# Autodesk Inventor assembly: 2015 Summer Worm Drive and Bevel Gear Box for Lift
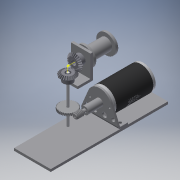
[picture p0: Inventor's stored thumbnail of the model, 180x180]
Saved by Autodesk Inventor 2016 (Build 200138000, 138)
## iProperties
Created: 2015-06-17
Part Number: 2015 Summer Worm Drive and Bevel Gear Box for Lift
Document SubType Name: Assembly
Designer: steele
Author: steele
## Documents named in this file (12)
- C:\snobotics\CAD\robSteele\Bevel Gearbox\2015 Summer Worm Drive and Bevel Gear Box for Lift.iam
- C:\snobotics\CAD\robSteele\Bevel Gearbox\baseForWormMotor.ipt
- C:\snobotics\CAD\robSteele\ipart Components\0_250 in diam aluminum rod\0_250 in diam aluminum rod-02.ipt
- C:\snobotics\CAD\robSteele\ipart Components\0_250 in diam aluminum rod.ipt
- C:\snobotics\CAD\partResources\Andy-Mark\motorMounts\AM 2488 CIM bracket.ipt
- C:\snobotics\CAD\partResources\Andy-Mark\Motors\AM 0255 MOT_CIM-Motor_217-2000.iam
- C:\snobotics\CAD\robSteele\CIM to 0_1875 Worm Gearn.ipt
- C:\snobotics\CAD\robSteele\Bevel Gearbox\g1036.ipt
- C:\snobotics\CAD\robSteele\Bevel Gearbox\LUHB.ipt
- C:\snobotics\CAD\robSteele\Bevel Gearbox\2015 Summer Bevel Gearbox\Angle Bracket for Bevel Gearbox.ipt
- C:\snobotics\CAD\robSteele\Bevel Gearbox\lift Hub.ipt
- C:\snobotics\CAD\robSteele\Bevel Gearbox\2015 Summer Bevel Gearbox\Design Accelerator\Bevel Gears1.iam
## Components (10 placed, 10 different names)
1. baseForWormMotor:1 — Insert:1, Mate:1, Flush:1, Flush:2, Insert:4
2. 0_250 in diam aluminum rod-02:1 — Insert:1, Tangent:1, Flush:3
3. AM 2488 CIM bracket:1 — Mate:1, Flush:1, Flush:2, Insert:2, Insert:3
4. AM 0255 MOT_CIM-Motor_217-2000:1 [sub-assembly] — Insert:2
5. CIM to 0_1875 Worm Gearn:1 — Insert:3, Insert:5
6. g1036:1 — Insert:4
7. LUHB:1 — Insert:5
8. Angle Bracket for Bevel Gearbox:1 — Tangent:1, Flush:3, Insert:6, Insert:7
9. lift Hub:1 — Insert:6
10. Bevel Gears:2 [sub-assembly] — Insert:7
## Relationships (12: Insert 7, Flush 3, Mate 1, Tangent 1)
- Insert:1: baseForWormMotor:1 ↔ 0_250 in diam aluminum rod-02:1
- Mate:1: baseForWormMotor:1 ↔ AM 2488 CIM bracket:1
- Flush:1: baseForWormMotor:1 ↔ AM 2488 CIM bracket:1
- Flush:2 (-101.6 mm): baseForWormMotor:1 ↔ AM 2488 CIM bracket:1
- Insert:2: AM 2488 CIM bracket:1 ↔ AM 0255 MOT_CIM-Motor_217-2000:1
- Insert:3: AM 2488 CIM bracket:1 ↔ CIM to 0_1875 Worm Gearn:1
- Insert:4 (42.8752 mm): baseForWormMotor:1 ↔ g1036:1
- Insert:5: CIM to 0_1875 Worm Gearn:1 ↔ LUHB:1
- Tangent:1: 0_250 in diam aluminum rod-02:1 ↔ Angle Bracket for Bevel Gearbox:1
- Flush:3 (19.05 mm): 0_250 in diam aluminum rod-02:1 ↔ Angle Bracket for Bevel Gearbox:1
- Insert:6 (2.54 mm): Angle Bracket for Bevel Gearbox:1 ↔ lift Hub:1
- Insert:7: Angle Bracket for Bevel Gearbox:1 ↔ Bevel Gears:2
